# Autodesk Inventor assembly: Product_TF Micro SD Card Memory Modul Arduino
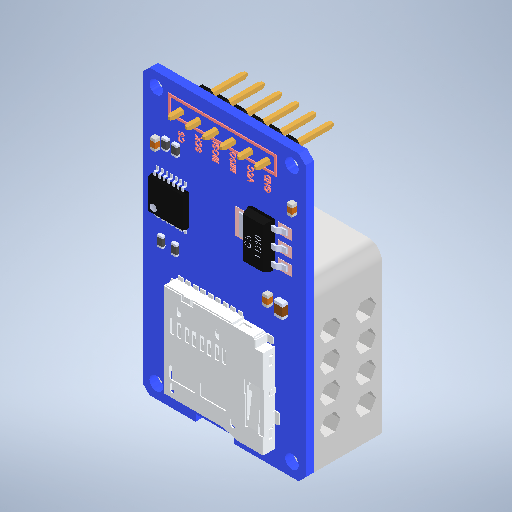
[picture p0: Inventor's stored thumbnail of the model, 512x512]
Saved by Autodesk Inventor 2025.2 (Build 292293000, 293)
## iProperties
Company: doctor
Created: 2021-05-16
Part Number: Product_TF Micro SD Card Memory Modul Arduino
Description: STEP AP214
Document SubType Name: Assembly
Designer: nugro
Title: Product_TF Micro SD Card Memory Modul Arduino.STEP
Author: mohamedamie
Revision Number: ANY
Sending System: SolidWorks 2012
Preprocessor: SwSTEP 2.0
## Documents named in this file (11)
- C:\Users\nugro\Documents\KiCad\Telemetry TAZ V1\Telemetry TAZ V1\3D Model\micro-sd-card-reader-module-1.snapshot.3\Product_TF Micro SD Card Memory Modul Arduino\Product_TF Micro SD Card Memory Modul Arduino\Pro.iam
- C:\Users\nugro\Documents\KiCad\Telemetry TAZ V1\Telemetry TAZ V1\3D Model\micro-sd-card-reader-module-1.snapshot.3\Product_TF Micro SD Card Memory Modul Arduino\Product_TF Micro SD Card Memory Modul Arduino\PCB.ipt
- C:\Users\nugro\Documents\KiCad\Telemetry TAZ V1\Telemetry TAZ V1\3D Model\micro-sd-card-reader-module-1.snapshot.3\Product_TF Micro SD Card Memory Modul Arduino\Product_TF Micro SD Card Memory Modul Arduino\slo.ipt
- C:\Users\nugro\Documents\KiCad\Telemetry TAZ V1\Telemetry TAZ V1\3D Model\micro-sd-card-reader-module-1.snapshot.3\Product_TF Micro SD Card Memory Modul Arduino\Product_TF Micro SD Card Memory Modul Arduino\nan.ipt
- C:\Users\nugro\Documents\KiCad\Telemetry TAZ V1\Telemetry TAZ V1\3D Model\micro-sd-card-reader-module-1.snapshot.3\Product_TF Micro SD Card Memory Modul Arduino\Product_TF Micro SD Card Memory Modul Arduino\res.ipt
- C:\Users\nugro\Documents\KiCad\Telemetry TAZ V1\Telemetry TAZ V1\3D Model\micro-sd-card-reader-module-1.snapshot.3\Product_TF Micro SD Card Memory Modul Arduino\Product_TF Micro SD Card Memory Modul Arduino\cap.ipt
- C:\Users\nugro\Documents\KiCad\Telemetry TAZ V1\Telemetry TAZ V1\3D Model\micro-sd-card-reader-module-1.snapshot.3\Product_TF Micro SD Card Memory Modul Arduino\Product_TF Micro SD Card Memory Modul Arduino\cap_1.ipt
- C:\Users\nugro\Documents\KiCad\Telemetry TAZ V1\Telemetry TAZ V1\3D Model\micro-sd-card-reader-module-1.snapshot.3\Product_TF Micro SD Card Memory Modul Arduino\Product_TF Micro SD Card Memory Modul Arduino\LVC.ipt
- C:\Users\nugro\Documents\KiCad\Telemetry TAZ V1\Telemetry TAZ V1\3D Model\micro-sd-card-reader-module-1.snapshot.3\Product_TF Micro SD Card Memory Modul Arduino\Product_TF Micro SD Card Memory Modul Arduino\Pin.iam
- C:\Users\nugro\Documents\KiCad\Telemetry TAZ V1\Telemetry TAZ V1\3D Model\micro-sd-card-reader-module-1.snapshot.3\Product_TF Micro SD Card Memory Modul Arduino\Product_TF Micro SD Card Memory Modul Arduino\Piè.ipt
- C:\Users\nugro\Documents\spacer sdcard m2.5.ipt
## Components (15 placed, 15 different names)
1. PCB_1 — Flush:1
2. slot_2
3. nano - reg_3
4. res_603_4
5. res_603_5
6. res_603_6
7. res_603_7
8. cap_603_8
9. cap_603_9
10. cap_603_10
11. cap_603_2_11
12. LVC125A_12
13. Pin Header Male 01x06 P2.54mm v1_13 [sub-assembly]
14. Pièce2_14
15. spacer sdcard m2.5:1 — Flush:1
## Relationships (1: Flush 1)
- Flush:1: PCB_1 ↔ spacer sdcard m2.5:1
